# Autodesk Inventor assembly: Assembly3
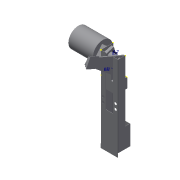
[picture p0: Inventor's stored thumbnail of the model, 180x180]
Saved by Autodesk Inventor 2019 (Build 230136000, 136)
## iProperties
Created: 2019-10-16
Part Number: Assembly3
Document SubType Name: Assembly
Designer: Admin
Author: Admin
## Documents named in this file (10)
- C:\Users\Admin\Documents\Assembly3.iam
- C:\Users\Admin\Documents\CAPPING SYSTEM DC MOTOR FIXING SYSTEM.ipt
- C:\Users\Admin\Documents\dc motor for capping system.ipt
- C:\Users\Admin\Documents\DC MOTOR NUT FOR CAPPING SYSTEM.ipt
- C:\Users\Admin\Documents\DC MOTOR NUT FOR CAPPING SYSTEM1.ipt
- C:\Users\Admin\Documents\crank for capping system.ipt
- C:\Users\Admin\Documents\shaft for capping system.ipt
- C:\Users\Admin\Documents\nut.ipt
- C:\Users\Admin\Documents\pusher.ipt
- C:\Users\Admin\Documents\crank shaft nut.ipt
## Components (10 placed, 9 different names)
1. CAPPING SYSTEM DC MOTOR FIXING SYSTEM:1 — Mate:1, Mate:2, Mate:4, Mate:15, Mate:16, Flush:1, Flush:2
2. dc motor for capping system:1 — Mate:1, Mate:2, Mate:3, Mate:5, Mate:6, Mate:7
3. DC MOTOR NUT FOR CAPPING SYSTEM:1 — Mate:3, Mate:4, Mate:8
4. DC MOTOR NUT FOR CAPPING SYSTEM1:1 — Mate:5, Mate:6
5. crank for capping system:1 — Mate:7, Mate:8, Mate:9, Mate:10, Mate:19, Mate:20
6. shaft for capping system:1 — Mate:9, Mate:10, Mate:17
7. pusher:1 — Mate:15, Mate:16, Mate:17, Mate:18, Mate:21, Mate:22
8. nut:2 — Mate:18
9. crank shaft nut:1 — Mate:19, Mate:20
10. crank shaft nut:2 — Mate:21, Mate:22
## Relationships (20: Mate 18, Flush 2)
- Mate:1: CAPPING SYSTEM DC MOTOR FIXING SYSTEM:1 ↔ dc motor for capping system:1
- Mate:2 (10.16 mm): CAPPING SYSTEM DC MOTOR FIXING SYSTEM:1 ↔ dc motor for capping system:1
- Mate:3: dc motor for capping system:1 ↔ DC MOTOR NUT FOR CAPPING SYSTEM:1
- Mate:4: CAPPING SYSTEM DC MOTOR FIXING SYSTEM:1 ↔ DC MOTOR NUT FOR CAPPING SYSTEM:1
- Mate:5: dc motor for capping system:1 ↔ DC MOTOR NUT FOR CAPPING SYSTEM1:1
- Mate:6: dc motor for capping system:1 ↔ DC MOTOR NUT FOR CAPPING SYSTEM1:1
- Mate:7: dc motor for capping system:1 ↔ crank for capping system:1
- Mate:8: DC MOTOR NUT FOR CAPPING SYSTEM:1 ↔ crank for capping system:1
- Mate:9: crank for capping system:1 ↔ shaft for capping system:1
- Mate:10: crank for capping system:1 ↔ shaft for capping system:1
- Mate:15: CAPPING SYSTEM DC MOTOR FIXING SYSTEM:1 ↔ pusher:1
- Mate:16: CAPPING SYSTEM DC MOTOR FIXING SYSTEM:1 ↔ pusher:1
- Flush:1: CAPPING SYSTEM DC MOTOR FIXING SYSTEM:1
- Flush:2: CAPPING SYSTEM DC MOTOR FIXING SYSTEM:1
- Mate:17: shaft for capping system:1 ↔ pusher:1
- Mate:18: pusher:1 ↔ nut:2
- Mate:19: crank for capping system:1 ↔ crank shaft nut:1
- Mate:20: crank for capping system:1 ↔ crank shaft nut:1
- Mate:21: pusher:1 ↔ crank shaft nut:2
- Mate:22: pusher:1 ↔ crank shaft nut:2
